# Autodesk Inventor assembly: eagle
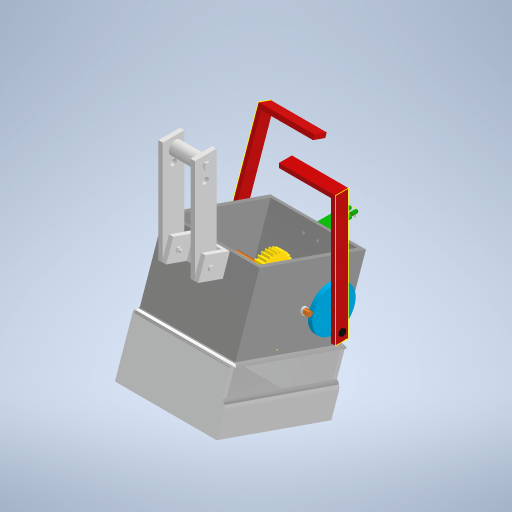
[picture p0: Inventor's stored thumbnail of the model, 512x512]
Saved by Autodesk Inventor 2023 (Build 270158000, 158)
## iProperties
Created: 2022-06-16
Part Number: eagle
Document SubType Name: Assembly
Designer: TRIVENI MAGADUM
Author: TRIVENI MAGADUM
## Documents named in this file (21)
- C:\Users\TRIVENI MAGADUM\Desktop\New folder\eagle.iam
- C:\Users\TRIVENI MAGADUM\Desktop\New folder\big gear.ipt
- C:\Users\TRIVENI MAGADUM\Desktop\New folder\container3.ipt
- C:\Users\TRIVENI MAGADUM\Desktop\New folder\DC MOTOR1.ipt
- C:\Users\TRIVENI MAGADUM\Desktop\New folder\Part4.ipt
- C:\Users\TRIVENI MAGADUM\Desktop\New folder\small gear.ipt
- C:\Users\TRIVENI MAGADUM\Desktop\New folder\cube.ipt
- C:\Users\TRIVENI MAGADUM\Desktop\New folder\Part1.ipt
- C:\Users\TRIVENI MAGADUM\Desktop\New folder\Part2.ipt
- C:\Users\TRIVENI MAGADUM\Desktop\New folder\Part3.ipt
- C:\Users\TRIVENI MAGADUM\Desktop\New folder\Screw 5 mm.ipt
- C:\Users\TRIVENI MAGADUM\Desktop\New folder\IR Sensor.ipt
- C:\Users\TRIVENI MAGADUM\Documents\container4.ipt
- C:\Users\TRIVENI MAGADUM\Desktop\New folder\Bolt 5mm.ipt
- E:\clamp.ipt
- E:\Stationary arm 2.ipt
- E:\Nylon rod.ipt
- E:\Stationary Arm\nut 5mm.ipt
- E:\Stationary Arm\Bolt 5mm.ipt
- E:\Stationary Arm\Screw 3mm.ipt
- E:\Stationary Arm\Bolt 3mm.ipt
## Components (45 placed, 19 different names)
1. container3:1 — Insert:1, Insert:2, Insert:3, Insert:4, Mate:1, Flush:1, Insert:14, Insert:15, Insert:21, Angle:1, Mate:2, Rigid:1, Insert:37, Insert:49, Insert:50
2. big gear:1 — Insert:5
3. big gear:2 — Insert:1, Rotation:1, Rotation:2
4. Part4:1 — Insert:2, Rotation:1, Rotation:2, Rotation:3
5. Part4:2 — Insert:4, Rotation:3, Rotational:1, Insert:7, Insert:11
6. small gear:2 — Insert:3
7. DC MOTOR1:2 — Tangent:1, Insert:5
8. cube:1 — Mate:1, Tangent:1, Flush:1
9. Part1:1 — Rotational:1
10. Part1:4 — Insert:7
11. Part1:5 — Insert:11
12. Part1:13 — Insert:14
13. Part1:15 — Insert:17
14. Part1:16 — Insert:15, Insert:16
15. Part2:1 — Insert:16, Insert:17, Insert:18, Mate:3
16. Part2:2 — Insert:22, Insert:23, Insert:24, Insert:36
17. Part1:17 — Insert:23
18. Part1:18 — Insert:21, Insert:22
19. Part1:19 — Insert:19, Insert:20
20. Part1:20 — Insert:18, Insert:19
21. Part3:1 — Insert:20, Insert:27
22. Part1:22 — Insert:25, Rotational:2
23. Part1:23 — Insert:24, Insert:25
24. Part3:2 — Rotational:2, Angle:1, Insert:35
25. Screw 5 mm:2 — Insert:27
26. IR Sensor:2 — Mate:2
27. container4:4 — Rigid:1
28. Bolt 5mm:1 — Mate:3
29. Bolt 5mm:2 — Insert:36
30. Screw 5 mm:3 — Insert:35
31. clamp:3
32. clamp:4 — Insert:37, Insert:38, Insert:39, Insert:44, Insert:46, Insert:47, Insert:48
33. Stationary arm 2:1 — Insert:38, Insert:40, Insert:45
34. Stationary arm 2:2 — Insert:39, Insert:41, Insert:42, Insert:43
35. Nylon rod:1 — Insert:40
36. nut 5mm:1 — Insert:41
37. Bolt 5mm:4 — Insert:42
38. Screw 3mm:1 — Insert:43
39. Screw 3mm:2 — Insert:44
40. Bolt 3mm:1 — Insert:45
41. Bolt 3mm:2 — Insert:46
42. Screw 3mm:3 — Insert:48
43. Screw 3mm:4 — Insert:47
44. Bolt 3mm:3 — Insert:49
45. Bolt 3mm:4 — Insert:50
## Relationships (48: Insert 36, RelateRotation 3, Mate 3, RevoluteJoint 2, Tangent 1, Flush 1, Angle 1, WeldJoint 1)
- Insert:1 (57 mm): container3:1 ↔ big gear:2
- Insert:2 (-10 mm): container3:1 ↔ Part4:1
- Insert:3 (57 mm): container3:1 ↔ small gear:2
- Insert:4 (-10 mm): container3:1 ↔ Part4:2
- Rotation:1 [RelateRotation] (20 ul): big gear:2 ↔ Part4:1
- Rotation:2 [RelateRotation] (1 ul): big gear:2 ↔ Part4:1
- Mate:1: container3:1 ↔ cube:1
- Tangent:1: DC MOTOR1:2 ↔ cube:1
- Insert:5 (-10 mm): big gear:1 ↔ DC MOTOR1:2
- Flush:1: container3:1 ↔ cube:1
- Rotation:3 [RelateRotation] (1 ul): Part4:1 ↔ Part4:2
- Rotational:1 [RevoluteJoint] (-11 mm): Part4:2 ↔ Part1:1
- Insert:7 (-13 mm): Part4:2 ↔ Part1:4
- Insert:11 (-11 mm): Part4:2 ↔ Part1:5
- Insert:14: container3:1 ↔ Part1:13
- Insert:15: container3:1 ↔ Part1:16
- Insert:16: Part1:16 ↔ Part2:1
- Insert:17: Part1:15 ↔ Part2:1
- Insert:18: Part2:1 ↔ Part1:20
- Insert:19: Part1:19 ↔ Part1:20
- Insert:20: Part1:19 ↔ Part3:1
- Insert:21: container3:1 ↔ Part1:18
- Insert:22: Part2:2 ↔ Part1:18
- Insert:23: Part2:2 ↔ Part1:17
- Insert:24: Part2:2 ↔ Part1:23
- Insert:25: Part1:22 ↔ Part1:23
- Rotational:2 [RevoluteJoint]: Part1:22 ↔ Part3:2
- Insert:27 (-15 mm): Part3:1 ↔ Screw 5 mm:2
- Angle:1 (0 deg): container3:1 ↔ Part3:2
- Mate:2: container3:1 ↔ IR Sensor:2
- Rigid:1 [WeldJoint]: container3:1 ↔ container4:4
- Mate:3 (-1 mm): Part2:1 ↔ Bolt 5mm:1
- Insert:35 (-14.5 mm): Part3:2 ↔ Screw 5 mm:3
- Insert:36 (-1 mm): Part2:2 ↔ Bolt 5mm:2
- Insert:37: container3:1 ↔ clamp:4
- Insert:38: clamp:4 ↔ Stationary arm 2:1
- Insert:39: clamp:4 ↔ Stationary arm 2:2
- Insert:40: Stationary arm 2:1 ↔ Nylon rod:1
- Insert:41 (-7.5 mm): Stationary arm 2:2 ↔ nut 5mm:1
- Insert:42: Stationary arm 2:2 ↔ Bolt 5mm:4
- Insert:43 (-15 mm): Stationary arm 2:2 ↔ Screw 3mm:1
- Insert:44 (-15 mm): clamp:4 ↔ Screw 3mm:2
- Insert:45: Stationary arm 2:1 ↔ Bolt 3mm:1
- Insert:46: clamp:4 ↔ Bolt 3mm:2
- Insert:47 (-16 mm): clamp:4 ↔ Screw 3mm:4
- Insert:48: clamp:4 ↔ Screw 3mm:3
- Insert:49: container3:1 ↔ Bolt 3mm:3
- Insert:50: container3:1 ↔ Bolt 3mm:4
